# Autodesk Inventor assembly: Cockpit_side_frame_MIR
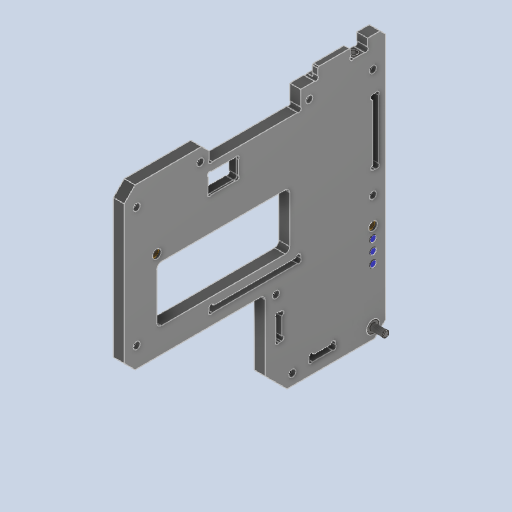
[picture p0: Inventor's stored thumbnail of the model, 512x512]
Saved by Autodesk Inventor 2022.3 (Build 263350000, 350)
## iProperties
Created: 2023-05-19
Part Number: Cockpit_side_frame_MIR
Document SubType Name: Assembly
Designer: Masato Kubotera
Author: Masato Kubotera
## Documents named in this file (6)
- C:\Users\Masato\Documents\Inventor\Inventor for CIT Brains\SUSTAINA-OP\UpperBody\Cockpit\Cockpit_side_frame_MIR.iam
- C:\Users\Masato\Documents\Inventor\Inventor for CIT Brains\SUSTAINA-OP\UpperBody\Cockpit\Cockpit_side_frame_MIR.ipt
- C:\Users\Masato\Documents\Inventor\Inventor for CIT Brains\SUSTAINA-OP\ReadyMade\Neodymium_magnet_Phi3_T3.ipt
- C:\Users\Masato\Documents\Inventor\Inventor for CIT Brains\SUSTAINA-OP\ReadyMade\InsertNut\UD-43040.ipt
- C:\Users\Masato\Documents\Inventor\Inventor for CIT Brains\SUSTAINA-OP\ReadyMade\InsertNut\IRU-304S.ipt
- C:\Users\Masato\Documents\Inventor\Inventor for CIT Brains\SUSTAINA-OP\ReadyMade\Spacer\BRU-305.ipt
## Components (8 placed, 5 different names)
1. Cockpit_side_frame_MIR:1 — Flush:1, Flush:2, Flush:3, Insert:1, Insert:2, Insert:3, Insert:4, Insert:5, Insert:6, Insert:7
2. Neodymium_magnet_Phi3_T3:1 — Insert:1
3. Neodymium_magnet_Phi3_T3:2 — Insert:2
4. Neodymium_magnet_Phi3_T3:3 — Insert:3
5. UD-43040:1 — Insert:4
6. IRU-304S:1 — Insert:6
7. BRU-305:1 — Insert:5
8. UD-43040:2 — Insert:7
## Relationships (10: Insert 7, Flush 3)
- Flush:1: Cockpit_side_frame_MIR:1
- Flush:2: Cockpit_side_frame_MIR:1
- Flush:3: Cockpit_side_frame_MIR:1
- Insert:1: Cockpit_side_frame_MIR:1 ↔ Neodymium_magnet_Phi3_T3:1
- Insert:2: Cockpit_side_frame_MIR:1 ↔ Neodymium_magnet_Phi3_T3:2
- Insert:3: Cockpit_side_frame_MIR:1 ↔ Neodymium_magnet_Phi3_T3:3
- Insert:4: Cockpit_side_frame_MIR:1 ↔ UD-43040:1
- Insert:5: Cockpit_side_frame_MIR:1 ↔ BRU-305:1
- Insert:6: Cockpit_side_frame_MIR:1 ↔ IRU-304S:1
- Insert:7: Cockpit_side_frame_MIR:1 ↔ UD-43040:2
